# Autodesk Inventor assembly: SawToothClip
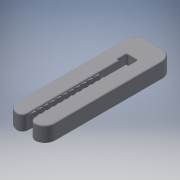
[picture p0: Inventor's stored thumbnail of the model, 180x180]
Saved by Autodesk Inventor 2016 (Build 200138000, 138)
## iProperties
Created: 2016-03-05
Part Number: SawToothClip
Document SubType Name: Assembly
Designer: yash
Author: yash
## Documents named in this file (3)
- C:\Users\yash\Documents\GitHub\HeadphoneBackClip\SawToothClip.iam
- C:\Users\yash\Documents\GitHub\HeadphoneBackClip\BaseClip.ipt
- C:\Users\yash\Documents\GitHub\HeadphoneBackClip\SawTeeth.ipt
## Components (2 placed, 2 different names)
1. BaseClip:1 — Mate:1, Mate:2, Mate:3
2. SawTeeth:1 — Mate:1, Mate:2, Mate:3
## Relationships (3: Mate 3)
- Mate:1: BaseClip:1 ↔ SawTeeth:1
- Mate:2: BaseClip:1 ↔ SawTeeth:1
- Mate:3: BaseClip:1 ↔ SawTeeth:1
